# Autodesk Inventor assembly: Estructura matriz centelladora
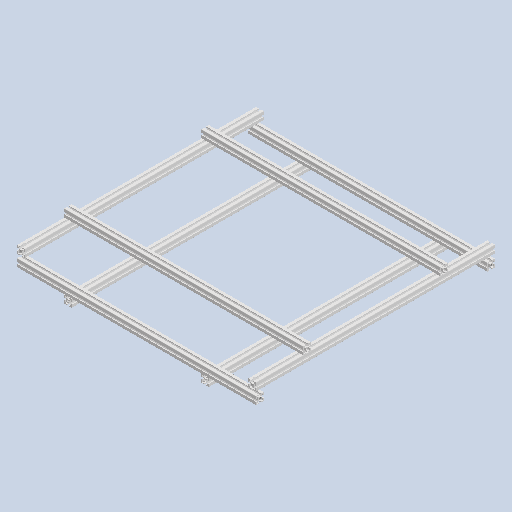
[picture p0: Inventor's stored thumbnail of the model, 512x512]
Saved by Autodesk Inventor 2024.2 (Build 282272000, 272)
## iProperties
Created: 2024-08-23
Part Number: Estructura matriz centelladora
Document SubType Name: Assembly
Designer: ja.restrepo1
Author: ja.restrepo1
## Documents named in this file (5)
- I:\MICROMECANICA\ALTAS ENERGIAS\Deteccion de Muones\Detectores\Detectores centelladores\Partes Detectores centelladores\PARTES DC\Perfileria 20x20 DC\SE estructura matriz centelladora.iam
- I:\MICROMECANICA\ALTAS ENERGIAS\Deteccion de Muones\Detectores\Detectores centelladores\Partes Detectores centelladores\PARTES DC\Perfileria 20x20 DC\Perfil 20X20 T.ipt
- I:\MICROMECANICA\ALTAS ENERGIAS\Deteccion de Muones\Detectores\Detectores centelladores\Partes Detectores centelladores\PARTES DC\Perfileria 20x20 DC\Perfil 20X20 T\Perfil 20X20 T-620BCAM5.ipt
- I:\MICROMECANICA\ALTAS ENERGIAS\Deteccion de Muones\Detectores\Detectores centelladores\Partes Detectores centelladores\PARTES DC\Perfileria 20x20 DC\Perfil 20X20 T\Perfil 20X20 T-620M5.ipt
- I:\MICROMECANICA\ALTAS ENERGIAS\Deteccion de Muones\Detectores\Detectores centelladores\Partes Detectores centelladores\PARTES DC\Perfileria 20x20 DC\Perfil 20X20 T\Perfil 20X20 T-620Ø5.ipt
## Components (8 placed, 3 different names)
1. Perfil 20X20 T-620BCAM5:1 — Nivelación:2, Nivelación:3, Coincidencia:2, Nivelación:10, Coincidencia:4, Nivelación:19, Coincidencia:10, Nivelación:22, Coincidencia:13
2. Perfil 20X20 T-620BCAM5:2 — Nivelación:1, Nivelación:3, Nivelación:8, Nivelación:9, Coincidencia:3, Coincidencia:4
3. Perfil 20X20 T-620M5:3 — Nivelación:6, Nivelación:7, Nivelación:8, Coincidencia:3, Nivelación:10, Nivelación:24, Coincidencia:14
4. Perfil 20X20 T-620M5:4 — Nivelación:5, Nivelación:7, Nivelación:9, Coincidencia:11
5. Perfil 20X20 T-620Ø5:5 — Nivelación:19, Coincidencia:9, Nivelación:20, Nivelación:21, Coincidencia:10, Nivelación:22, Coincidencia:11
6. Perfil 20X20 T-620Ø5:6 — Coincidencia:9, Nivelación:20, Nivelación:21
7. Perfil 20X20 T-620Ø5:7 — Nivelación:23, Coincidencia:12, Nivelación:24, Nivelación:25, Coincidencia:13, Coincidencia:14
8. Perfil 20X20 T-620Ø5:8 — Nivelación:23, Coincidencia:12, Nivelación:25
## Relationships (25: Flush 16, Mate 9)
- Nivelación:1 [Flush]: Perfil 20X20 T-620BCAM5:2
- Nivelación:2 [Flush]: Perfil 20X20 T-620BCAM5:1
- Nivelación:3 [Flush]: Perfil 20X20 T-620BCAM5:1 ↔ Perfil 20X20 T-620BCAM5:2
- Coincidencia:2 [Mate] (5 mm): Perfil 20X20 T-620BCAM5:1
- Nivelación:5 [Flush]: Perfil 20X20 T-620M5:4
- Nivelación:6 [Flush]: Perfil 20X20 T-620M5:3
- Nivelación:7 [Flush]: Perfil 20X20 T-620M5:3 ↔ Perfil 20X20 T-620M5:4
- Nivelación:8 [Flush]: Perfil 20X20 T-620BCAM5:2 ↔ Perfil 20X20 T-620M5:3
- Nivelación:9 [Flush]: Perfil 20X20 T-620BCAM5:2 ↔ Perfil 20X20 T-620M5:4
- Coincidencia:3 [Mate] (10 mm): Perfil 20X20 T-620BCAM5:2 ↔ Perfil 20X20 T-620M5:3
- Nivelación:10 [Flush]: Perfil 20X20 T-620BCAM5:1 ↔ Perfil 20X20 T-620M5:3
- Coincidencia:4 [Mate] (570 mm): Perfil 20X20 T-620BCAM5:1 ↔ Perfil 20X20 T-620BCAM5:2
- Nivelación:19 [Flush]: Perfil 20X20 T-620BCAM5:1 ↔ Perfil 20X20 T-620Ø5:5
- Coincidencia:9 [Mate] (330 mm): Perfil 20X20 T-620Ø5:5 ↔ Perfil 20X20 T-620Ø5:6
- Nivelación:20 [Flush]: Perfil 20X20 T-620Ø5:5 ↔ Perfil 20X20 T-620Ø5:6
- Nivelación:21 [Flush]: Perfil 20X20 T-620Ø5:5 ↔ Perfil 20X20 T-620Ø5:6
- Coincidencia:10 [Mate]: Perfil 20X20 T-620BCAM5:1 ↔ Perfil 20X20 T-620Ø5:5
- Nivelación:22 [Flush]: Perfil 20X20 T-620BCAM5:1 ↔ Perfil 20X20 T-620Ø5:5
- Coincidencia:11 [Mate] (100 mm): Perfil 20X20 T-620M5:4 ↔ Perfil 20X20 T-620Ø5:5
- Nivelación:23 [Flush]: Perfil 20X20 T-620Ø5:7 ↔ Perfil 20X20 T-620Ø5:8
- Coincidencia:12 [Mate] (330 mm): Perfil 20X20 T-620Ø5:7 ↔ Perfil 20X20 T-620Ø5:8
- Nivelación:24 [Flush]: Perfil 20X20 T-620M5:3 ↔ Perfil 20X20 T-620Ø5:7
- Nivelación:25 [Flush]: Perfil 20X20 T-620Ø5:7 ↔ Perfil 20X20 T-620Ø5:8
- Coincidencia:13 [Mate] (100 mm): Perfil 20X20 T-620BCAM5:1 ↔ Perfil 20X20 T-620Ø5:7
- Coincidencia:14 [Mate]: Perfil 20X20 T-620M5:3 ↔ Perfil 20X20 T-620Ø5:7
